# Autodesk Inventor assembly: Plattenzusammensetzung
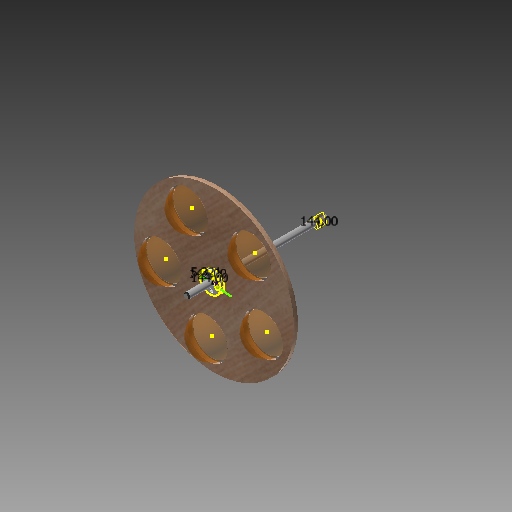
[picture p0: Inventor's stored thumbnail of the model, 512x512]
Saved by Autodesk Inventor 2018 (Build 220112000, 112)
## iProperties
Created: 2017-10-13
Part Number: Plattenzusammensetzung
Material: Generisch
Document SubType Name: Assembly
Designer: Dominik
Author: Dominik
## Documents named in this file (11)
- C:\Users\Dominik\Desktop\Diplomarbeit\fuettr_prototype\Mechanical\Inventorskizzen\Plattenzusammensetzung.iam
- C:\Users\Dominik\Desktop\Diplomarbeit\fuettr_prototype\Mechanical\Inventorskizzen\Drehplatte_Rahmenvorrrichtung.ipt
- C:\Users\Dominik\Desktop\Diplomarbeit\fuettr_prototype\Mechanical\Inventorskizzen\Futterschüssel_innen.ipt
- C:\Users\Dominik\Desktop\Diplomarbeit\fuettr_prototype\Mechanical\Inventorskizzen\Welle.ipt
- C:\Users\Dominik\Desktop\Diplomarbeit\fuettr_prototype\Mechanical\Inventorskizzen\Flansch.ipt
- C:\Users\Julian\Documents\Inventor\Content Center Files\R2018\de-DE\DIN 711\DIN 711 - 512 01 - 12 x 28 x 11.ipt
- C:\Users\Dominik\Desktop\Diplomarbeit\fuettr_prototype\Mechanical\Inventorskizzen\Plattenzusammensetzung\AIP\FEA\cfy8r9bk0.fins
- C:\Users\Dominik\Desktop\Diplomarbeit\fuettr_prototype\Mechanical\Inventorskizzen\Plattenzusammensetzung\AIP\FEA\cfy8r9bkw.fsat
- C:\Users\Dominik\Desktop\Diplomarbeit\fuettr_prototype\Mechanical\Inventorskizzen\Plattenzusammensetzung\AIP\FEA\cfy8r9bkw.ftes
- C:\Users\Dominik\Desktop\Diplomarbeit\fuettr_prototype\Mechanical\Inventorskizzen\Plattenzusammensetzung\AIP\FEA\cfy8r9bls.fwiz
- C:\Users\Dominik\Desktop\Diplomarbeit\fuettr_prototype\Mechanical\Inventorskizzen\Plattenzusammensetzung\AIP\FEA\cfy8r9c80.fmsh
## Components (9 placed, 5 different names)
1. Drehplatte_Rahmenvorrrichtung:1 — Passend:1, Passend:3, Passend:4, Passend:5, Passend:6, Passend:7, Passend:8, Passend:9, Passend:10, Passend:11, Passend:12, Passend:18, Passend:19
2. Futterschüssel_innen:1 — Passend:3, Passend:4
3. Welle:1 — Passend:1, Passend:17, Passend:20, Drehbar:1
4. Futterschüssel_innen:2 — Passend:5, Passend:6
5. Futterschüssel_innen:3 — Passend:11, Passend:12
6. Futterschüssel_innen:4 — Passend:9, Passend:10
7. Futterschüssel_innen:5 — Passend:7, Passend:8
8. Flansch:1 — Passend:17, Passend:18, Passend:19, Passend:20
9. DIN 711 512 01 - 12 x 28 x 11:1 — Drehbar:1
## Relationships (16: Mate 15, RevoluteJoint 1)
- Passend:1 [Mate]: Drehplatte_Rahmenvorrrichtung:1 ↔ Welle:1
- Passend:3 [Mate]: Drehplatte_Rahmenvorrrichtung:1 ↔ Futterschüssel_innen:1
- Passend:4 [Mate]: Drehplatte_Rahmenvorrrichtung:1 ↔ Futterschüssel_innen:1
- Passend:5 [Mate]: Drehplatte_Rahmenvorrrichtung:1 ↔ Futterschüssel_innen:2
- Passend:6 [Mate]: Drehplatte_Rahmenvorrrichtung:1 ↔ Futterschüssel_innen:2
- Passend:7 [Mate]: Drehplatte_Rahmenvorrrichtung:1 ↔ Futterschüssel_innen:5
- Passend:8 [Mate]: Drehplatte_Rahmenvorrrichtung:1 ↔ Futterschüssel_innen:5
- Passend:9 [Mate]: Drehplatte_Rahmenvorrrichtung:1 ↔ Futterschüssel_innen:4
- Passend:10 [Mate]: Drehplatte_Rahmenvorrrichtung:1 ↔ Futterschüssel_innen:4
- Passend:11 [Mate]: Drehplatte_Rahmenvorrrichtung:1 ↔ Futterschüssel_innen:3
- Passend:12 [Mate]: Drehplatte_Rahmenvorrrichtung:1 ↔ Futterschüssel_innen:3
- Passend:17 [Mate]: Welle:1 ↔ Flansch:1
- Passend:18 [Mate]: Drehplatte_Rahmenvorrrichtung:1 ↔ Flansch:1
- Passend:19 [Mate]: Drehplatte_Rahmenvorrrichtung:1 ↔ Flansch:1
- Passend:20 [Mate]: Welle:1 ↔ Flansch:1
- Drehbar:1 [RevoluteJoint]: Welle:1 ↔ DIN 711 512 01 - 12 x 28 x 11:1
## Named parameters: sa_0 = 1800, sa_2 = 900
note: some values were not read from the file. Shown as the stored number, unit unknown: "sa_0", "sa_2".
